# Autodesk Inventor assembly: Сборка 3_4 вариант
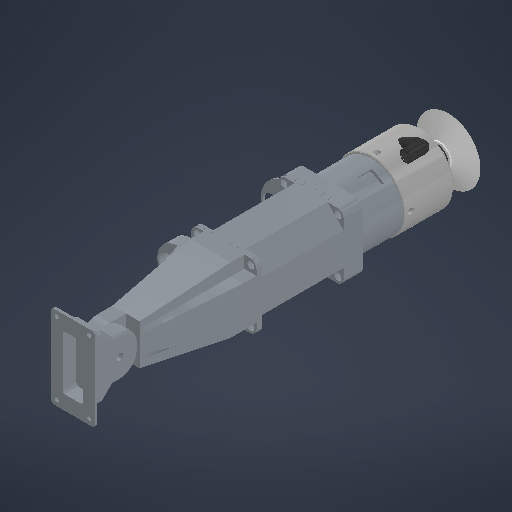
[picture p0: Inventor's stored thumbnail of the model, 512x512]
Saved by Autodesk Inventor 2026 (Build 300175000, 175)
## iProperties
Company: UNSPECIFIED
Created: 1900-01-01
Part Number: Сборка 3_4 вариант
Description: STEP AP214
Document SubType Name: Assembly
Designer: kvm13
Title: Ñáîðêà 3_3 âàðèàíò
Author: UNSPECIFIED
Revision Number: ANYUNSPECIFIED
Sending System: C3D Toolkit
Preprocessor: C3D Converter
## Documents named in this file (7)
- C:\Users\kvm13\Desktop\MIK-nozzle\3D Форсунка фрикад\Сборка форсунки.iam
- C:\Users\kvm13\Desktop\MIK-nozzle\3D Форсунка фрикад\Сборка 3_4 вариант\Сборка 3_4 вариант\Деталь.ipt
- C:\Users\kvm13\Desktop\MIK-nozzle\3D Форсунка фрикад\Сборка 3_4 вариант\Сборка 3_4 вариант\Деталь_2.ipt
- C:\Users\kvm13\Desktop\MIK-nozzle\3D Форсунка фрикад\Сборка 3_4 вариант\Сборка 3_4 вариант\Деталь_3.ipt
- C:\Users\kvm13\Desktop\MIK-nozzle\3D Форсунка фрикад\Байонет ванны.ipt
- C:\Users\kvm13\Desktop\MIK-nozzle\3D Форсунка фрикад\Статор диска.ipt
- C:\Users\kvm13\Desktop\MIK-nozzle\3D Форсунка фрикад\Корпус форсунки 1\Корпус форсунки 1\Корпус форсунки 1.iam
## Components (7 placed, 4 different names)
1. ANY — Жесткий:1, Жесткий:3
2. ANY:2
3. ANY:3
4. ANY:4
5. Байонет ванны:1 — Жесткий:1, Жесткий:2
6. Статор диска:1 — Жесткий:2
7. Корпус форсунки 1:1 [sub-assembly] — Жесткий:3
## Relationships (3: WeldJoint 3)
- Жесткий:1 [WeldJoint] (1.25 mm): ANY ↔ Байонет ванны:1
- Жесткий:2 [WeldJoint]: Байонет ванны:1 ↔ Статор диска:1
- Жесткий:3 [WeldJoint]: ANY ↔ Корпус форсунки 1:1
